(part 1 of 2)
# Autodesk Inventor assembly: 1103 Robot - Base2
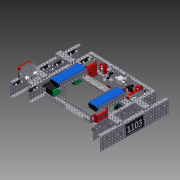
[picture p0: Inventor's stored thumbnail of the model, 180x180]
Saved by Autodesk Inventor 2012 (Build 160160000, 160)
## iProperties
Created: 2011-08-15
Part Number: 1103 Robot - Base2
Document SubType Name: Assembly
Designer: Dakota.Bayer
Author: Dakota.Bayer
## Documents named in this file (50)
- C:\Users\Wade\Documents\1103 Robot - CAD Assembly\1103 Chassis.iam
- C:\Users\Wade\Documents\1103 Robot - CAD Assembly\5 x 25.ipt
- C:\Users\Wade\Documents\1103 Robot - CAD Assembly\Flat Bearing Block.ipt
- C:\Users\Wade\Documents\1103 Robot - CAD Assembly\5 x 24.ipt
- C:\Users\Wade\Documents\1103 Robot - CAD Assembly\Bearing Block.iam
- C:\Users\Wade\Documents\1103 Robot - CAD Assembly\2 x 6.ipt
- C:\Users\Wade\Documents\1103 Robot - CAD Assembly\1103 Custom Chassis.ipt
- C:\Users\Wade\Documents\1103 Robot - CAD Assembly\2 x 25.ipt
- C:\Users\Wade\Documents\1103 Robot - CAD Assembly\4 Slotted Angle.ipt
- C:\Users\Wade\Documents\1103 Robot - CAD Assembly\4 x 6 cut.ipt
- C:\Users\Wade\Documents\1103 Robot - CAD Assembly\.5'' Screw & Nylock Nut.iam
- C:\Users\Wade\Documents\1103 Robot - CAD Assembly\2x .5'' Screw & Nylock Nut.iam
- C:\Users\Wade\Documents\24C VEX CAD Files\Screws & Nuts\Screw 8-32 x 0.500''-Silver.ipt
- C:\Users\Wade\Documents\24C VEX CAD Files\Screws & Nuts\Screw 6-32 x 0.500''-Silver.ipt
- C:\Users\Wade\Documents\24C VEX CAD Files\Screws & Nuts\Nut 8-32 Nylock.ipt
- C:\Users\Wade\Documents\24C VEX CAD Files\Washers & Spacers\Spacer (Nylon), 0.375''.ipt
- C:\Users\Wade\Documents\24C VEX CAD Files\Standoffs & Couplers\Standoff 0.50''.ipt
- C:\Users\Wade\Documents\24C VEX CAD Files\Screws & Nuts\Screw 8-32 x 0.250''-Silver.ipt
- C:\Users\Wade\Documents\24C VEX CAD Files\Screws & Nuts\Nut 8-32 Keps.ipt
- C:\Users\Wade\Documents\24C VEX CAD Files\Screws & Nuts\Screw 8-32 x 0.750''-Silver.ipt
- C:\Users\Wade\Documents\24C VEX CAD Files\Screws & Nuts\Screw 8-32 x 0.375''-Silver.ipt
- C:\Users\Wade\Documents\1103 Robot - CAD Assembly\.375'' Screw & Nylock Nut.iam
- C:\Users\Wade\Documents\24C VEX CAD Files\Motors & Sensors\2-Wire Motor 393-Without Wire.iam
- C:\Users\Wade\Documents\24C VEX CAD Files\Motors & Sensors\Ultrasonic Range Finder (Sensor).iam
- C:\Users\Wade\Documents\1103 Robot - CAD Assembly\VEX-HINGE-1 RevA_1.ipt
- C:\Users\Wade\Documents\1103 Robot - CAD Assembly\VEX-HINGE-PIN_1.ipt
- C:\Users\Wade\Documents\1103 Robot - CAD Assembly\VEX-HINGE-1 RevA 4x.ipt
- C:\Users\Wade\Documents\1103 Robot - CAD Assembly\VEX-HINGE-PIN 4x.ipt
- C:\Users\Wade\Documents\24C VEX CAD Files\Washers & Spacers\Spacer (Nylon), 0.125''.ipt
- C:\Users\Wade\Documents\1103 Robot - CAD Assembly\Drivetrain Encoder.iam
- C:\Users\Wade\Documents\24C VEX CAD Files\Motors & Sensors\Line Follower Sensor (Line Tracker)-Parts\Custom1x4 Mount.ipt
- C:\Users\Wade\Documents\24C VEX CAD Files\Other Parts\On-Off Switch.iam
- C:\Users\Wade\Documents\1103 Robot - CAD Assembly\5 x 25 Custom.ipt
- C:\Users\Wade\Documents\1103 Robot - CAD Assembly\Input Potentiometer.iam
- C:\Users\Wade\Documents\24C VEX CAD Files\Other Parts\Regulator Body.ipt
- C:\Users\Wade\Documents\24C VEX CAD Files\Other Parts\Regulator Nut.ipt
- C:\Users\Wade\Documents\24C VEX CAD Files\Other Parts\Tier Pump Fitting Nut.ipt
- C:\Users\Wade\Documents\24C VEX CAD Files\Other Parts\Tire Pump Fitting.ipt
- C:\Users\Wade\Documents\24C VEX CAD Files\Other Parts\Fitting for Cylinders.ipt
- C:\Users\Wade\Documents\24C VEX CAD Files\Metal Plates\Metal L (3x2) .ipt
- C:\Users\Wade\Documents\24C VEX CAD Files\Other Parts\Pneumatic Cylinder Mount.ipt
- C:\Users\Wade\Documents\1103 Robot - CAD Assembly\1103 ID Plate (with hardware).iam
- C:\Users\Wade\Documents\24C VEX CAD Files\Metal Plates\Plate 6x3.ipt
- C:\Users\Wade\Documents\24C VEX CAD Files\Metal C-Channels\Aluminum L-Channel 1x5x2.ipt
- C:\Users\Wade\Documents\24C VEX CAD Files\Metal Plates\Plate 4x3.ipt
- C:\Users\Wade\Documents\24C VEX CAD Files\Metal Angles\Angle 2x2x10.ipt
- C:\Users\Wade\Documents\24C VEX CAD Files\Other Parts\7.2V (Robot Battery) NiMH 3000mAh.ipt
- C:\Users\Wade\Documents\24C VEX CAD Files\Motors & Sensors\Line Follower Sensor (Line Tracker).iam
- C:\Users\Wade\Documents\24C VEX CAD Files\Washers & Spacers\Washer, Delrin.ipt
- C:\Users\Wade\Documents\24C VEX CAD Files\Screws & Nuts\Screw 8-32 x 0.875''-Silver.ipt
## Components (259 placed, 49 different names)
1. 5 x 25:2 — Mate:3, Mate:22, Mate:42, Mate:57, Mate:74, Flush:1, Flush:2, Flush:18, Flush:19, Mate:255, Flush:20, Flush:21, Flush:22, Flush:23, Flush:58, Flush:59, Mate:326, Mate:327, Mate:330, Mate:583, Mate:584, Angle:6, Mate:599, Mate:600, Mate:699
2. Flat Bearing Block:1 — Mate:3, Mate:324, Mate:325, Mate:698
3. .5'' Screw & Nylock Nut:3 [sub-assembly] — Mate:327, Mate:328
4. Flat Bearing Block:2 — Mate:22, Mate:328, Mate:329
5. Screw 8-32 x 0.500''-Silver:1 — Mate:366
6. Flat Bearing Block:3 — Mate:42, Mate:356, Mate:357
7. Screw 8-32 x 0.500''-Silver:2 — Mate:367
8. Screw 8-32 x 0.500''-Silver:3 — Mate:365
9. Flat Bearing Block:4 — Mate:57, Mate:358, Mate:359
10. Screw 8-32 x 0.500''-Silver:4 — Mate:364
11. Screw 8-32 x 0.500''-Silver:5 — Mate:363
12. Flat Bearing Block:5 — Mate:74, Mate:360, Mate:361
13. Screw 8-32 x 0.500''-Silver:6 — Mate:362
14. 5 x 24:1 — Flush:1, Flush:2, Mate:98, Mate:99, Mate:104, Mate:109, Mate:121, Flush:3, Flush:4, Mate:253, Mate:254, Mate:318, Flush:58, Flush:59, Mate:322, Tangent:152, Tangent:153, Tangent:154, Tangent:155, Tangent:156, Mate:422, Tangent:186, Mate:432, Tangent:190, Tangent:191, Mate:452, Flush:67, Mate:481, Mate:482, Flush:68, Mate:485, Tangent:220, Mate:598, Flush:555, Flush:556, Mate:695, Mate:696, Mate:697, Mate:701, Mate:703, Mate:704, Mate:705, Mate:706
15. Bearing Block:1 [sub-assembly] — Mate:98, Tangent:152, Tangent:153, Tangent:154
16. Flat Bearing Block:7 — Mate:99, Mate:319, Mate:320, Mate:323, Mate:695, Mate:696, Mate:698, Mate:700
17. Flat Bearing Block:8 — Mate:104, Mate:478, Mate:479, Mate:702
18. Screw 6-32 x 0.500''-Silver:2 — Mate:703, Mate:704, Mate:707
19. Screw 6-32 x 0.500''-Silver:3
20. Screw 6-32 x 0.500''-Silver:4
21. Flat Bearing Block:9 — Mate:109
22. 2-Wire Motor 393-Without Wire:1 [sub-assembly]
23. 2-Wire Motor 393-Without Wire:2 [sub-assembly] — Mate:478, Mate:480, Mate:702, Mate:707
24. 5 x 25 Custom:1 — Mate:121, Flush:3, Flush:4, Mate:122, Flush:5, Flush:6, Mate:430, Tangent:187, Mate:431, Tangent:188, Tangent:189, Mate:483, Mate:489, Mate:511, Mate:512, Mate:523, Angle:2, Mate:525, Mate:526, Mate:527, Mate:528, Mate:529, Mate:530, Mate:531, Mate:532, Mate:535, Mate:536, Angle:3, Mate:538, Mate:539, Mate:540, Mate:542, Angle:4, Flush:71, Mate:545, Flush:546, Mate:546, Flush:547, Flush:548, Mate:551, Mate:553, Mate:574, Mate:576, Mate:682, Angle:10, Mate:732
25. 5 x 24:2 — Mate:122, Flush:5, Flush:6, Mate:123, Mate:133, Mate:139, Flush:7, Flush:8, Mate:242, Mate:244, Mate:250, Flush:34, Flush:57, Tangent:157, Tangent:158, Tangent:159, Tangent:160, Tangent:161, Tangent:162, Mate:333, Mate:433, Tangent:192, Tangent:193, Mate:486, Tangent:221, Tangent:222, Tangent:223, Mate:488, Mate:514, Mate:515, Mate:516, Mate:518, Flush:553, Mate:596, Flush:554, Angle:7, Mate:708, Mate:709, Mate:710, Mate:711
26. .5'' Screw & Nylock Nut:5 [sub-assembly] — Mate:332, Mate:333
27. Screw 8-32 x 0.500''-Silver:8 — Mate:335
28. Flat Bearing Block:10 — Mate:123, Mate:332, Mate:334, Mate:700
29. Flat Bearing Block:11 — Mate:250
30. Screw 6-32 x 0.500''-Silver:5
31. Screw 6-32 x 0.500''-Silver:6
32. Bearing Block:2 [sub-assembly] — Mate:133, Tangent:157, Tangent:158, Tangent:159
33. Flat Bearing Block:12 — Mate:244, Mate:712
34. Screw 6-32 x 0.500''-Silver:7 — Mate:708, Mate:709
35. Bearing Block:3 [sub-assembly] — Mate:139, Tangent:160, Tangent:161, Tangent:162
36. 2-Wire Motor 393-Without Wire:3 [sub-assembly] — Mate:249, Mate:712
37. 2-Wire Motor 393-Without Wire:4 [sub-assembly]
38. 5 x 25:4 — Flush:7, Flush:8, Mate:207, Mate:213, Mate:219, Mate:224, Mate:229, Mate:241, Rotation:2, Flush:56, Mate:581, Mate:582, Angle:5, Mate:585
39. Screw 8-32 x 0.500''-Silver:9 — Mate:354
40. Screw 8-32 x 0.500''-Silver:10 — Mate:355
41. Flat Bearing Block:13 — Mate:207, Mate:352, Mate:353
42. Screw 8-32 x 0.500''-Silver:11 — Mate:346
43. Screw 8-32 x 0.500''-Silver:12 — Mate:347
44. Flat Bearing Block:14 — Mate:213, Mate:344, Mate:345
45. Screw 8-32 x 0.500''-Silver:13 — Mate:350
46. Screw 8-32 x 0.500''-Silver:14 — Mate:351
47. Flat Bearing Block:15 — Mate:219, Rotation:2, Mate:348, Mate:349
48. Screw 8-32 x 0.500''-Silver:15 — Mate:342
49. Screw 8-32 x 0.500''-Silver:16 — Mate:343
50. Flat Bearing Block:16 — Mate:224, Mate:340, Mate:341
51. Screw 8-32 x 0.500''-Silver:17 — Mate:336
52. Screw 8-32 x 0.500''-Silver:18 — Mate:337
53. Flat Bearing Block:17 — Mate:229, Mate:338, Mate:339
54. Standoff 0.50'':1 — Mate:381
55. Standoff 0.50'':2 — Mate:383
56. Standoff 0.50'':3 — Mate:380
57. Standoff 0.50'':4 — Mate:382
58. Standoff 0.50'':5 — Mate:372
59. Standoff 0.50'':6 — Mate:374
60. Standoff 0.50'':7 — Mate:375
61. Standoff 0.50'':8 — Mate:373
62. 2 x 6:1 — Mate:255, Flush:20, Flush:21, Mate:368, Mate:369
63. 2 x 6:2 — Mate:254, Flush:18, Flush:19, Mate:370, Mate:371
64. 2 x 6:3 — Mate:241, Flush:57, Mate:378, Mate:379
65. 2 x 6:4 — Mate:242, Mate:376, Mate:377
66. Screw 6-32 x 0.500''-Silver:8 — Mate:249, Mate:710, Mate:711
67. 1103 Custom Chassis:1 — Mate:253, Flush:22, Flush:23, Flush:56, Tangent:171, Tangent:172, Mate:423, Tangent:173, Tangent:174, Mate:424, Mate:425, Tangent:175, Tangent:176, Tangent:177, Mate:426, Mate:427, Tangent:178, Tangent:179, Tangent:180, Tangent:181, Mate:428, Mate:429, Tangent:182, Tangent:183, Tangent:184, Tangent:185, Tangent:207, Mate:611, Flush:557, Flush:558, Mate:612, Flush:559, Flush:560, Mate:613, Mate:614, Mate:615, Mate:616, Mate:617, Mate:618, Mate:619, Mate:621, Mate:622, Mate:623, Mate:624
68. 2 x 25:1 — Flush:34, Mate:434, Mate:435, Flush:62, Flush:63, Flush:64, Flush:65, Mate:448, Mate:449, Tangent:199, Tangent:200, Tangent:201, Tangent:202, Mate:450, Mate:451, Tangent:203, Tangent:204, Tangent:205, Tangent:206, Mate:452, Flush:67, Mate:453, Mate:456, Mate:457, Mate:458, Mate:459, Mate:468, Mate:469, Mate:470, Mate:471, Mate:472
69. Standoff 0.50'':9 — Mate:386
70. Standoff 0.50'':10 — Mate:387
71. 4 Slotted Angle:1 — Mate:384, Mate:385, Mate:418, Mate:419
72. Spacer (Nylon), 0.375'':1 — Mate:416
73. Spacer (Nylon), 0.375'':2 — Mate:417
74. 4 x 6 cut:1 — Mate:414, Mate:415
75. Ultrasonic Range Finder (Sensor):1 [sub-assembly]
76. Standoff 0.50'':11 — Mate:390
77. Standoff 0.50'':12 — Mate:391
78. 4 Slotted Angle:2 — Mate:388, Mate:389, Mate:410, Mate:411
79. Spacer (Nylon), 0.375'':3 — Mate:408
80. Spacer (Nylon), 0.375'':4 — Mate:409
81. 4 x 6 cut:2 — Mate:406, Mate:407
82. Ultrasonic Range Finder (Sensor):2 [sub-assembly]
83. Bearing Block:4 [sub-assembly] — Mate:318, Tangent:155, Tangent:156, Mate:701
84. .5'' Screw & Nylock Nut:1 [sub-assembly] — Mate:319, Mate:320
85. .5'' Screw & Nylock Nut:2 [sub-assembly] — Mate:322, Mate:323, Mate:697
86. 2x .5'' Screw & Nylock Nut:1 [sub-assembly] — Mate:324, Mate:325, Mate:326, Mate:699
87. .5'' Screw & Nylock Nut:4 [sub-assembly] — Mate:329, Mate:330
88. Nut 8-32 Nylock:1 — Mate:334, Mate:335
89. Nut 8-32 Nylock:2 — Mate:336, Mate:338
90. Nut 8-32 Nylock:3 — Mate:337, Mate:339
91. Nut 8-32 Nylock:4 — Mate:340, Mate:342
92. Nut 8-32 Nylock:5 — Mate:341, Mate:343
93. Nut 8-32 Nylock:6 — Mate:345, Mate:347
94. Nut 8-32 Nylock:7 — Mate:344, Mate:346
95. Nut 8-32 Nylock:8 — Mate:348, Mate:351
96. Nut 8-32 Nylock:9 — Mate:349, Mate:350
97. Nut 8-32 Nylock:10 — Mate:352, Mate:355
98. Nut 8-32 Nylock:11 — Mate:353, Mate:354
99. Nut 8-32 Nylock:12 — Mate:356, Mate:366
100. Nut 8-32 Nylock:13 — Mate:357, Mate:367
101. Nut 8-32 Nylock:14 — Mate:358, Mate:364
102. Nut 8-32 Nylock:15 — Mate:359, Mate:365
103. Nut 8-32 Nylock:16 — Mate:361, Mate:363
104. Nut 8-32 Nylock:17 — Mate:360, Mate:362
105. Screw 8-32 x 0.250''-Silver:1 — Mate:368, Mate:372
106. Screw 8-32 x 0.250''-Silver:2 — Mate:369, Mate:373
107. Screw 8-32 x 0.250''-Silver:3 — Mate:371, Mate:375
108. Screw 8-32 x 0.250''-Silver:4 — Mate:370, Mate:374
109. Screw 8-32 x 0.250''-Silver:5 — Mate:379, Mate:381
110. Screw 8-32 x 0.250''-Silver:6 — Mate:378, Mate:380
111. Screw 8-32 x 0.250''-Silver:7 — Mate:377, Mate:382
112. Screw 8-32 x 0.250''-Silver:8 — Mate:376, Mate:383
113. Screw 8-32 x 0.250''-Silver:9 — Mate:384, Mate:386
114. Screw 8-32 x 0.250''-Silver:10 — Mate:385, Mate:387
115. Screw 8-32 x 0.250''-Silver:11 — Mate:388, Mate:391
116. Screw 8-32 x 0.250''-Silver:12 — Mate:389, Mate:390
117. Screw 8-32 x 0.375''-Silver:2
118. Screw 8-32 x 0.375''-Silver:1
119. Nut 8-32 Keps:1
120. Nut 8-32 Keps:2
121. Nut 8-32 Keps:3
122. Screw 8-32 x 0.375''-Silver:4
123. Nut 8-32 Keps:4
124. Screw 8-32 x 0.375''-Silver:3
125. Screw 8-32 x 0.750''-Silver:1 — Mate:406, Mate:408, Mate:413
126. Screw 8-32 x 0.750''-Silver:2 — Mate:407, Mate:409, Mate:412
127. Nut 8-32 Nylock:18 — Mate:410, Mate:413
128. Nut 8-32 Nylock:19 — Mate:411, Mate:412
129. Screw 8-32 x 0.750''-Silver:3 — Mate:414, Mate:416, Mate:421
130. Screw 8-32 x 0.750''-Silver:4 — Mate:415, Mate:417, Mate:420
131. Nut 8-32 Nylock:20 — Mate:418, Mate:421
132. Nut 8-32 Nylock:21 — Mate:419, Mate:420
133. .375'' Screw & Nylock Nut:1 [sub-assembly] — Tangent:171, Tangent:172, Mate:422
134. .375'' Screw & Nylock Nut:2 [sub-assembly] — Mate:425, Tangent:175, Tangent:176
135. .375'' Screw & Nylock Nut:3 [sub-assembly] — Mate:423, Tangent:173, Tangent:174
136. .375'' Screw & Nylock Nut:4 [sub-assembly] — Mate:424, Tangent:177, Tangent:207
137. .375'' Screw & Nylock Nut:5 [sub-assembly] — Mate:426, Tangent:178, Tangent:179
138. .375'' Screw & Nylock Nut:6 [sub-assembly] — Mate:427, Tangent:180, Tangent:181
139. .375'' Screw & Nylock Nut:7 [sub-assembly] — Mate:428, Tangent:184, Tangent:185
140. .375'' Screw & Nylock Nut:8 [sub-assembly] — Mate:429, Tangent:182, Tangent:183
141. .375'' Screw & Nylock Nut:9 [sub-assembly] — Mate:430, Tangent:186, Tangent:187
142. .375'' Screw & Nylock Nut:10 [sub-assembly] — Mate:431, Tangent:188, Tangent:189
143. .375'' Screw & Nylock Nut:11 [sub-assembly] — Mate:432, Tangent:190, Tangent:191
144. .375'' Screw & Nylock Nut:12 [sub-assembly] — Mate:433, Tangent:192, Tangent:193
145. VEX-HINGE-1 RevA_1:1 — Mate:434, Mate:437, Flush:60, Flush:62, Flush:63, Flush:66, Tangent:210, Tangent:211, Tangent:212, Tangent:213, Tangent:214, Tangent:215, Mate:464, Mate:465, Mate:466
146. VEX-HINGE-PIN_1:1 — Mate:437, Flush:60
147. VEX-HINGE-1 RevA 4x:1 — Mate:435, Mate:436, Flush:61, Flush:64, Flush:65, Tangent:208, Tangent:209, Mate:455, Tangent:216, Tangent:217, Mate:467
148. VEX-HINGE-PIN 4x:1 — Mate:436, Flush:61
149. Screw 8-32 x 0.500''-Silver:23 — Mate:463, Mate:464, Mate:473
150. Screw 8-32 x 0.500''-Silver:21 — Mate:461, Mate:466, Mate:475
151. Screw 8-32 x 0.500''-Silver:20 — Mate:460, Mate:467, Mate:476
152. Screw 8-32 x 0.500''-Silver:22 — Mate:462, Mate:465, Mate:474
153. Screw 8-32 x 0.500''-Silver:19 — Mate:454, Mate:455, Mate:477
154. .375'' Screw & Nylock Nut:18 [sub-assembly] — Mate:448, Tangent:199, Tangent:200
155. .375'' Screw & Nylock Nut:19 [sub-assembly] — Mate:449, Tangent:201, Tangent:202
156. .375'' Screw & Nylock Nut:20 [sub-assembly] — Mate:450, Tangent:203, Tangent:204
157. .375'' Screw & Nylock Nut:21 [sub-assembly] — Mate:451, Tangent:205, Tangent:206
158. Spacer (Nylon), 0.125'':1 — Mate:453, Tangent:208, Tangent:209, Mate:454
159. Spacer (Nylon), 0.125'':2 — Mate:456, Tangent:216, Tangent:217, Mate:460
160. Spacer (Nylon), 0.125'':3 — Mate:457, Tangent:214, Tangent:215, Mate:461
161. Spacer (Nylon), 0.125'':4 — Mate:458, Tangent:212, Tangent:213, Mate:462
162. Spacer (Nylon), 0.125'':5 — Mate:459, Tangent:210, Tangent:211, Mate:463
163. Nut 8-32 Nylock:22 — Mate:468, Mate:473
164. Nut 8-32 Nylock:23 — Mate:469, Mate:474
165. Nut 8-32 Nylock:24 — Mate:470, Mate:475
166. Nut 8-32 Nylock:25 — Mate:471, Mate:476
167. Nut 8-32 Nylock:26 — Mate:472, Mate:477
168. Screw 6-32 x 0.500''-Silver:9 — Mate:479, Mate:480, Mate:481, Mate:705, Mate:706
169. Drivetrain Encoder:1 [sub-assembly] — Mate:482, Flush:68, Mate:483, Mate:484
170. Drivetrain Encoder:2 [sub-assembly] — Mate:487, Mate:488, Mate:489
171. Bearing Block:5 [sub-assembly] — Mate:484, Mate:485, Tangent:220
172. Bearing Block:6 [sub-assembly] — Mate:486, Tangent:221, Tangent:222, Tangent:223, Mate:487
173. Screw 8-32 x 0.250''-Silver:13 — Mate:509, Mate:510, Mate:682
174. Screw 8-32 x 0.375''-Silver:5 — Mate:507, Mate:681, Mate:687, Mate:731
175. Screw 8-32 x 0.375''-Silver:6 — Mate:504, Mate:683, Mate:684, Mate:686, Mate:729
176. Screw 8-32 x 0.375''-Silver:7 — Mate:503, Mate:688, Mate:690, Mate:730
177. Nut 8-32 Nylock:27 — Mate:504, Mate:505, Mate:683, Mate:685
178. Nut 8-32 Nylock:28 — Mate:503, Mate:506, Mate:691
179. Custom1x4 Mount:1 — Mate:505, Mate:506, Mate:508, Mate:512, Mate:681, Mate:684, Mate:685, Mate:689, Mate:690, Mate:691, Mate:692, Mate:693
180. Line Follower Sensor (Line Tracker):1 [sub-assembly] — Mate:686, Mate:693, Angle:8, Mate:729
181. Line Follower Sensor (Line Tracker):2 [sub-assembly] — Mate:688, Mate:689, Angle:9, Mate:730, Mate:731
182. Line Follower Sensor (Line Tracker):3 [sub-assembly] — Mate:687, Mate:692, Angle:8, Angle:9, Angle:10
183. Standoff 0.50'':13 — Mate:507, Mate:508, Mate:509, Mate:510, Mate:511
184. Line Follower Sensor (Line Tracker):4 [sub-assembly] — Mate:679, Mate:680, Angle:7
185. Screw 8-32 x 0.250''-Silver:14 — Mate:514, Mate:515, Mate:516, Mate:517
186. Standoff 0.50'':14 — Mate:517, Mate:518, Mate:521, Mate:680
187. Screw 8-32 x 0.375''-Silver:8 — Mate:521, Mate:679
188. On-Off Switch:1 [sub-assembly] — Mate:523, Angle:2, Mate:732
189. Input Potentiometer:1 [sub-assembly] — Mate:525, Mate:527, Mate:528, Mate:529
190. Input Potentiometer:2 [sub-assembly] — Mate:526, Mate:530, Mate:531, Mate:532
191. Regulator Body:1 — Mate:535, Mate:537, Angle:3, Mate:538, Mate:544, Mate:694
192. Regulator Nut:1 — Mate:536, Mate:537
193. Tier Pump Fitting Nut:1 — Mate:541, Mate:542
194. Tire Pump Fitting:1 — Mate:539, Mate:540, Mate:541, Angle:4
195. Fitting for Cylinders:1 — Mate:544, Mate:694
196. Metal L (3x2) :1 — Flush:71, Mate:545, Flush:546, Mate:554, Mate:555, Mate:560, Flush:551, Flush:552, Mate:573
197. Metal L (3x2) :2 — Mate:546, Flush:547, Flush:548, Mate:550, Mate:552, Mate:559, Flush:549, Flush:550, Mate:575
198. .375'' Screw & Nylock Nut:22 [sub-assembly] — Mate:553, Mate:554, Mate:555
199. .375'' Screw & Nylock Nut:24 [sub-assembly] — Mate:550, Mate:551, Mate:552
200. Pneumatic Cylinder Mount:1 — Mate:559, Flush:549, Flush:550, Mate:567, Mate:568, Mate:569, Mate:570, Mate:571, Mate:572, Mate:717, Mate:718, Mate:719, Mate:721, Mate:722, Mate:724
201. Pneumatic Cylinder Mount:2 — Mate:560, Flush:551, Flush:552, Mate:561, Mate:562, Mate:566, Mate:713, Mate:714, Mate:715, Mate:725, Mate:727, Mate:728
202. Screw 8-32 x 0.500''-Silver:25 — Mate:567, Mate:568, Mate:571, Mate:578
203. Screw 8-32 x 0.375''-Silver:9 — Mate:579
204. Screw 8-32 x 0.500''-Silver:27 — Mate:561, Mate:562, Mate:566, Mate:580
205. Screw 8-32 x 0.375''-Silver:10 — Mate:569, Mate:570, Mate:572, Mate:577
206. Nut 8-32 Nylock:29 — Mate:573, Mate:579
207. Nut 8-32 Nylock:30 — Mate:574, Mate:580
208. Nut 8-32 Nylock:31 — Mate:575, Mate:577
209. Nut 8-32 Nylock:32 — Mate:576, Mate:578
210. 1103 ID Plate (with hardware):1 [sub-assembly] — Mate:581, Mate:582, Angle:5
211. 1103 ID Plate (with hardware):2 [sub-assembly] — Mate:583, Mate:584, Angle:6
212. Plate 6x3:1 — Mate:585, Flush:553, Flush:554, Mate:586, Mate:587, Mate:588, Mate:589, Mate:590, Mate:591, Mate:592, Mate:594, Mate:595, Mate:597, Mate:593
213. .375'' Screw & Nylock Nut:25 [sub-assembly] — Mate:586, Mate:587, Mate:588
214. .375'' Screw & Nylock Nut:26 [sub-assembly] — Mate:589, Mate:590, Mate:591
215. .375'' Screw & Nylock Nut:27 [sub-assembly] — Mate:595, Mate:596, Mate:597
216. .375'' Screw & Nylock Nut:28 [sub-assembly] — Mate:592, Mate:593, Mate:594
217. Plate 6x3:2 — Mate:598, Flush:555, Flush:556, Mate:601, Mate:602, Mate:603, Mate:604, Mate:605, Mate:606, Mate:607, Mate:608, Mate:609, Mate:610
218. .375'' Screw & Nylock Nut:29 [sub-assembly] — Mate:599, Mate:600, Mate:601
219. .375'' Screw & Nylock Nut:30 [sub-assembly] — Mate:602, Mate:603, Mate:604
220. .375'' Screw & Nylock Nut:31 [sub-assembly] — Mate:608, Mate:609, Mate:610
221. .375'' Screw & Nylock Nut:32 [sub-assembly] — Mate:605, Mate:606, Mate:607
222. Aluminum L-Channel 1x5x2:1 — Mate:611, Flush:557, Flush:558, Flush:561, Mate:625, Flush:562, Mate:667, Mate:668
223. Aluminum L-Channel 1x5x2:2 — Mate:612, Flush:559, Flush:560, Mate:620, Mate:626, Flush:627, Flush:628, Mate:669, Mate:670, Mate:677, Mate:678
224. .375'' Screw & Nylock Nut:33 [sub-assembly] — Mate:613, Mate:614, Mate:615
225. .375'' Screw & Nylock Nut:34 [sub-assembly] — Mate:616, Mate:617, Mate:618
226. .375'' Screw & Nylock Nut:35 [sub-assembly] — Mate:619, Mate:620, Mate:621
227. .375'' Screw & Nylock Nut:36 [sub-assembly] — Mate:622, Mate:623, Mate:624
228. Plate 4x3:1 — Flush:561, Mate:625, Flush:562, Mate:627, Flush:629, Flush:630, Mate:628, Flush:631, Flush:632, Mate:663
229. Plate 4x3:2 — Mate:626, Flush:627, Flush:628, Mate:629, Flush:633, Flush:634, Mate:630, Flush:635, Flush:636, Mate:641
230. Angle 2x2x10:1 — Mate:627, Flush:629, Flush:630, Mate:631, Mate:632, Mate:633, Mate:646, Mate:647, Mate:648, Mate:656, Flush:637, Mate:659, Mate:660, Mate:661, Mate:662, Mate:664
231. Angle 2x2x10:2 — Mate:628, Flush:631, Flush:632, Mate:634, Mate:635, Mate:636, Mate:643, Mate:644, Mate:645, Mate:655
232. Angle 2x2x10:3 — Mate:629, Flush:633, Flush:634, Mate:637, Mate:638, Mate:639, Mate:649, Mate:650, Mate:651
233. Angle 2x2x10:4 — Mate:630, Flush:635, Flush:636, Mate:640, Mate:642, Mate:652, Mate:653, Mate:654, Mate:657, Mate:658, Flush:638, Mate:671, Mate:672, Mate:673, Mate:674
234. .375'' Screw & Nylock Nut:37 [sub-assembly] — Mate:631, Mate:632, Mate:633
235. .375'' Screw & Nylock Nut:38 [sub-assembly] — Mate:634, Mate:635, Mate:636
236. .375'' Screw & Nylock Nut:39 [sub-assembly] — Mate:637, Mate:638, Mate:639
237. .375'' Screw & Nylock Nut:40 [sub-assembly] — Mate:640, Mate:641, Mate:642
238. .375'' Screw & Nylock Nut:41 [sub-assembly] — Mate:646, Mate:647, Mate:648
239. .375'' Screw & Nylock Nut:42 [sub-assembly] — Mate:643, Mate:644, Mate:645
240. .375'' Screw & Nylock Nut:43 [sub-assembly] — Mate:652, Mate:653, Mate:654
241. .375'' Screw & Nylock Nut:44 [sub-assembly] — Mate:649, Mate:650, Mate:651
242. 7.2V (Robot Battery) NiMH 3000mAh:1 — Mate:655, Mate:656, Flush:637
243. 7.2V (Robot Battery) NiMH 3000mAh:2 — Mate:657, Mate:658, Flush:638
244. Screw 8-32 x 0.375''-Silver:11 — Mate:659, Mate:660, Mate:661, Mate:666
245. Screw 8-32 x 0.375''-Silver:12 — Mate:662, Mate:663, Mate:664, Mate:665
246. Nut 8-32 Nylock:33 — Mate:666, Mate:667
247. Nut 8-32 Nylock:34 — Mate:665, Mate:668
248. Screw 8-32 x 0.375''-Silver:13 — Mate:672, Mate:673, Mate:674, Mate:676
249. Nut 8-32 Nylock:35 — Mate:675, Mate:677
250. Screw 8-32 x 0.375''-Silver:14 — Mate:669, Mate:670, Mate:671, Mate:675
251. Nut 8-32 Nylock:36 — Mate:676, Mate:678
252. Washer, Delrin:1 — Mate:713, Mate:715, Mate:716
253. Washer, Delrin:2 — Mate:714, Mate:716
254. Washer, Delrin:3 — Mate:718, Mate:719, Mate:720
255. Washer, Delrin:4 — Mate:717, Mate:720
256. Nut 8-32 Nylock:37 — Mate:723, Mate:724
257. Screw 8-32 x 0.875''-Silver:1 — Mate:721, Mate:722, Mate:723
258. Nut 8-32 Nylock:38 — Mate:726, Mate:727
259. Screw 8-32 x 0.875''-Silver:2 — Mate:725, Mate:726, Mate:728
## Relationships (704: Mate 477, Tangent 157, Flush 60, Angle 9, RelateRotation 1)
- Mate:3: 5 x 25:2 ↔ Flat Bearing Block:1
- Mate:22: 5 x 25:2 ↔ Flat Bearing Block:2
- [Mate]: 5 x 25:2 ↔ Screw 8-32 x 0.500''-Silver:2
- [Tangent] (0.2286 mm): 5 x 25:2 ↔ Screw 8-32 x 0.500''-Silver:2
- [Tangent] (0.2286 mm): 5 x 25:2 ↔ Screw 8-32 x 0.500''-Silver:2
- [Mate]: 5 x 25:2 ↔ Screw 8-32 x 0.500''-Silver:1
- [Tangent] (0.2286 mm): 5 x 25:2 ↔ Screw 8-32 x 0.500''-Silver:1
- [Tangent] (0.2286 mm): 5 x 25:2 ↔ Screw 8-32 x 0.500''-Silver:1
- Mate:42: 5 x 25:2 ↔ Flat Bearing Block:3
- [Mate]: Screw 8-32 x 0.500''-Silver:1 ↔ Flat Bearing Block:3
- [Mate]: Flat Bearing Block:3 ↔ Screw 8-32 x 0.500''-Silver:2
- Mate:57: 5 x 25:2 ↔ Flat Bearing Block:4
- [Mate]: 5 x 25:2 ↔ Screw 8-32 x 0.500''-Silver:4
- [Tangent] (0.2286 mm): 5 x 25:2 ↔ Screw 8-32 x 0.500''-Silver:4
- [Tangent] (0.2286 mm): 5 x 25:2 ↔ Screw 8-32 x 0.500''-Silver:4
- [Mate]: 5 x 25:2 ↔ Screw 8-32 x 0.500''-Silver:3
- [Tangent] (0.2286 mm): 5 x 25:2 ↔ Screw 8-32 x 0.500''-Silver:3
- [Tangent] (0.2286 mm): 5 x 25:2 ↔ Screw 8-32 x 0.500''-Silver:3
- [Mate]: Flat Bearing Block:4 ↔ Screw 8-32 x 0.500''-Silver:4
- [Mate]: Screw 8-32 x 0.500''-Silver:3 ↔ Flat Bearing Block:4
- Mate:74: 5 x 25:2 ↔ Flat Bearing Block:5
- [Mate] (-1.524 mm): 5 x 25:2 ↔ Screw 8-32 x 0.500''-Silver:5
- [Tangent] (0.2286 mm): 5 x 25:2 ↔ Screw 8-32 x 0.500''-Silver:5
- [Tangent] (0.2286 mm): 5 x 25:2 ↔ Screw 8-32 x 0.500''-Silver:5
- [Mate] (-1.524 mm): 5 x 25:2 ↔ Screw 8-32 x 0.500''-Silver:6
- [Tangent] (0.2286 mm): 5 x 25:2 ↔ Screw 8-32 x 0.500''-Silver:6
- [Tangent] (0.2286 mm): 5 x 25:2 ↔ Screw 8-32 x 0.500''-Silver:6
- [Mate]: Screw 8-32 x 0.500''-Silver:5 ↔ Flat Bearing Block:5
- [Mate]: Flat Bearing Block:5 ↔ Screw 8-32 x 0.500''-Silver:6
- Flush:1: 5 x 25:2 ↔ 5 x 24:1
- Flush:2: 5 x 25:2 ↔ 5 x 24:1
- Mate:98: 5 x 24:1 ↔ Bearing Block:1
- Mate:99: 5 x 24:1 ↔ Flat Bearing Block:7
- Mate:104: 5 x 24:1 ↔ Flat Bearing Block:8
- [Mate]: 5 x 24:1 ↔ Screw 6-32 x 0.500''-Silver:2
- Mate:109: 5 x 24:1 ↔ Flat Bearing Block:9
- [Mate]: 5 x 24:1 ↔ Screw 6-32 x 0.500''-Silver:3
- [Mate]: 5 x 24:1 ↔ Screw 6-32 x 0.500''-Silver:4
- [Mate]: Screw 6-32 x 0.500''-Silver:3 ↔ Flat Bearing Block:9
- [Mate]: Screw 6-32 x 0.500''-Silver:4 ↔ Flat Bearing Block:9
- [Mate]: Flat Bearing Block:9 ↔ 2-Wire Motor 393-Without Wire:1
- [Mate]: Screw 6-32 x 0.500''-Silver:3 ↔ 2-Wire Motor 393-Without Wire:1
- [Mate]: Screw 6-32 x 0.500''-Silver:4 ↔ 2-Wire Motor 393-Without Wire:1
- [Mate]: Flat Bearing Block:8 ↔ 2-Wire Motor 393-Without Wire:2
- Mate:121: 5 x 24:1 ↔ 5 x 25 Custom:1
- Flush:3: 5 x 24:1 ↔ 5 x 25 Custom:1
- Flush:4: 5 x 24:1 ↔ 5 x 25 Custom:1
- Mate:122: 5 x 25 Custom:1 ↔ 5 x 24:2
- Flush:5: 5 x 25 Custom:1 ↔ 5 x 24:2
- Flush:6: 5 x 25 Custom:1 ↔ 5 x 24:2
- Mate:123: 5 x 24:2 ↔ Flat Bearing Block:10
- [Tangent] (0.2286 mm): 5 x 24:2 ↔ Screw 8-32 x 0.500''-Silver:8
- [Tangent] (0.2286 mm): 5 x 24:2 ↔ Screw 8-32 x 0.500''-Silver:8
- [Mate]: Screw 8-32 x 0.500''-Silver:8 ↔ Flat Bearing Block:10
- [Mate]: 5 x 24:2 ↔ Screw 6-32 x 0.500''-Silver:6
- [Mate]: 5 x 24:2 ↔ Screw 6-32 x 0.500''-Silver:5
- [Mate]: Flat Bearing Block:11 ↔ Screw 6-32 x 0.500''-Silver:5
- [Mate]: Flat Bearing Block:11 ↔ Screw 6-32 x 0.500''-Silver:6
- Mate:133: 5 x 24:2 ↔ Bearing Block:2
- [Mate]: 5 x 24:2 ↔ Screw 6-32 x 0.500''-Silver:7
- Mate:139: 5 x 24:2 ↔ Bearing Block:3
- [Mate]: Flat Bearing Block:12 ↔ 2-Wire Motor 393-Without Wire:3
- [Mate]: Flat Bearing Block:11 ↔ 2-Wire Motor 393-Without Wire:4
- Flush:7: 5 x 24:2 ↔ 5 x 25:4
- Flush:8: 5 x 24:2 ↔ 5 x 25:4
- Mate:207: 5 x 25:4 ↔ Flat Bearing Block:13
- [Mate]: 5 x 25:4 ↔ Screw 8-32 x 0.500''-Silver:9
- [Tangent] (0.2286 mm): 5 x 25:4 ↔ Screw 8-32 x 0.500''-Silver:9
- [Tangent] (0.2286 mm): 5 x 25:4 ↔ Screw 8-32 x 0.500''-Silver:9
- [Mate]: 5 x 25:4 ↔ Screw 8-32 x 0.500''-Silver:10
- [Tangent] (0.2286 mm): 5 x 25:4 ↔ Screw 8-32 x 0.500''-Silver:10
- [Tangent] (0.2286 mm): 5 x 25:4 ↔ Screw 8-32 x 0.500''-Silver:10
- [Mate]: Screw 8-32 x 0.500''-Silver:9 ↔ Flat Bearing Block:13
- [Mate]: Screw 8-32 x 0.500''-Silver:10 ↔ Flat Bearing Block:13
- [Mate]: 5 x 25:4 ↔ Screw 8-32 x 0.500''-Silver:11
- Mate:213: 5 x 25:4 ↔ Flat Bearing Block:14
- [Mate]: 5 x 25:4 ↔ Screw 8-32 x 0.500''-Silver:12
- [Tangent] (0.2286 mm): 5 x 25:4 ↔ Screw 8-32 x 0.500''-Silver:11
- [Tangent] (0.2286 mm): 5 x 25:4 ↔ Screw 8-32 x 0.500''-Silver:11
- [Tangent] (0.2286 mm): 5 x 25:4 ↔ Screw 8-32 x 0.500''-Silver:12
- [Tangent] (0.2286 mm): 5 x 25:4 ↔ Screw 8-32 x 0.500''-Silver:12
- [Mate]: Screw 8-32 x 0.500''-Silver:11 ↔ Flat Bearing Block:14
- [Mate]: Screw 8-32 x 0.500''-Silver:12 ↔ Flat Bearing Block:14
- [Mate] (-1.524 mm): 5 x 25:4 ↔ Screw 8-32 x 0.500''-Silver:13
- [Mate] (-1.524 mm): 5 x 25:4 ↔ Screw 8-32 x 0.500''-Silver:14
- Mate:219: 5 x 25:4 ↔ Flat Bearing Block:15
- [Tangent] (0.2286 mm): 5 x 25:4 ↔ Screw 8-32 x 0.500''-Silver:13
- [Tangent] (0.2286 mm): 5 x 25:4 ↔ Screw 8-32 x 0.500''-Silver:13
- [Tangent] (0.2286 mm): 5 x 25:4 ↔ Screw 8-32 x 0.500''-Silver:14
- [Tangent] (0.2286 mm): 5 x 25:4 ↔ Screw 8-32 x 0.500''-Silver:14
- [Mate]: Screw 8-32 x 0.500''-Silver:13 ↔ Flat Bearing Block:15
- [Mate]: Screw 8-32 x 0.500''-Silver:14 ↔ Flat Bearing Block:15
- [Mate]: 5 x 25:4 ↔ Screw 8-32 x 0.500''-Silver:15
- [Mate]: 5 x 25:4 ↔ Screw 8-32 x 0.500''-Silver:16
- Mate:224: 5 x 25:4 ↔ Flat Bearing Block:16
- [Tangent] (0.2286 mm): 5 x 25:4 ↔ Screw 8-32 x 0.500''-Silver:15
- [Tangent] (0.2286 mm): 5 x 25:4 ↔ Screw 8-32 x 0.500''-Silver:15
- [Tangent] (0.2286 mm): 5 x 25:4 ↔ Screw 8-32 x 0.500''-Silver:16
- [Tangent] (0.2286 mm): 5 x 25:4 ↔ Screw 8-32 x 0.500''-Silver:16
- [Mate]: Screw 8-32 x 0.500''-Silver:15 ↔ Flat Bearing Block:16
- [Mate]: Screw 8-32 x 0.500''-Silver:16 ↔ Flat Bearing Block:16
- [Mate]: 5 x 25:4 ↔ Screw 8-32 x 0.500''-Silver:18
- [Mate]: 5 x 25:4 ↔ Screw 8-32 x 0.500''-Silver:17
- Mate:229: 5 x 25:4 ↔ Flat Bearing Block:17
- [Tangent] (0.2286 mm): 5 x 25:4 ↔ Screw 8-32 x 0.500''-Silver:17
- [Tangent] (0.2286 mm): 5 x 25:4 ↔ Screw 8-32 x 0.500''-Silver:17
- [Tangent] (0.2286 mm): 5 x 25:4 ↔ Screw 8-32 x 0.500''-Silver:18
- [Tangent] (0.2286 mm): 5 x 25:4 ↔ Screw 8-32 x 0.500''-Silver:18
- [Mate]: Screw 8-32 x 0.500''-Silver:17 ↔ Flat Bearing Block:17
- [Mate]: Screw 8-32 x 0.500''-Silver:18 ↔ Flat Bearing Block:17
- [Mate]: 5 x 25:4 ↔ Standoff 0.50'':1
- [Mate]: 5 x 25:4 ↔ Standoff 0.50'':3
- [Mate]: 5 x 25:2 ↔ Standoff 0.50'':6
- [Mate]: 5 x 24:1 ↔ Standoff 0.50'':7
- [Mate]: 5 x 24:1 ↔ Standoff 0.50'':5
- [Mate]: 5 x 25:2 ↔ Standoff 0.50'':8
- Mate:241: 5 x 25:4 ↔ 2 x 6:3
- Mate:242: 5 x 24:2 ↔ 2 x 6:4
- Mate:244: 5 x 24:2 ↔ Flat Bearing Block:12
- [Mate]: Flat Bearing Block:12 ↔ 2-Wire Motor 393-Without Wire:3
- [Mate]: Flat Bearing Block:12 ↔ Screw 6-32 x 0.500''-Silver:7
- [Mate]: 5 x 24:2 ↔ Screw 6-32 x 0.500''-Silver:8
- Mate:249: 2-Wire Motor 393-Without Wire:3 ↔ Screw 6-32 x 0.500''-Silver:8
- [Tangent] (0.4572 mm): 5 x 24:2 ↔ Screw 6-32 x 0.500''-Silver:6
- [Tangent] (0.4572 mm): 5 x 24:2 ↔ Screw 6-32 x 0.500''-Silver:6
- Mate:250: 5 x 24:2 ↔ Flat Bearing Block:11
- [Tangent] (0.4572 mm): 5 x 24:2 ↔ Screw 6-32 x 0.500''-Silver:5
- [Mate]: Screw 6-32 x 0.500''-Silver:6 ↔ 2-Wire Motor 393-Without Wire:4
- [Mate]: Screw 6-32 x 0.500''-Silver:5 ↔ 2-Wire Motor 393-Without Wire:4
- [Tangent] (0.4572 mm): 5 x 24:1 ↔ Screw 6-32 x 0.500''-Silver:3
- [Tangent] (0.4572 mm): 5 x 24:1 ↔ Screw 6-32 x 0.500''-Silver:3
- [Tangent] (0.4572 mm): 5 x 24:1 ↔ Screw 6-32 x 0.500''-Silver:4
- Mate:253: 5 x 24:1 ↔ 1103 Custom Chassis:1
- Mate:254: 5 x 24:1 ↔ 2 x 6:2
- Flush:18: 5 x 25:2 ↔ 2 x 6:2
- Flush:19: 5 x 25:2 ↔ 2 x 6:2
- Mate:255: 5 x 25:2 ↔ 2 x 6:1
- Flush:20: 5 x 25:2 ↔ 2 x 6:1
- Flush:21: 5 x 25:2 ↔ 2 x 6:1
- Flush:22: 5 x 25:2 ↔ 1103 Custom Chassis:1
- Flush:23: 5 x 25:2 ↔ 1103 Custom Chassis:1
- Flush:34: 5 x 24:2 ↔ 2 x 25:1
- [Mate]: 5 x 24:1 ↔ Standoff 0.50'':9
- [Mate]: 5 x 24:1 ↔ Standoff 0.50'':10
- [Tangent] (0.2286 mm): 5 x 24:1 ↔ Standoff 0.50'':9
- [Tangent] (0.2286 mm): 5 x 24:1 ↔ Standoff 0.50'':9
- [Tangent] (0.2286 mm): 5 x 24:1 ↔ Standoff 0.50'':10
- [Tangent] (0.2286 mm): 5 x 24:1 ↔ Standoff 0.50'':10
- [Mate]: Standoff 0.50'':9 ↔ 4 Slotted Angle:1
- [Tangent] (0.2286 mm): Standoff 0.50'':10 ↔ 4 Slotted Angle:1
- [Tangent] (0.2286 mm): Standoff 0.50'':9 ↔ 4 Slotted Angle:1
- [Tangent] (0.2286 mm): Standoff 0.50'':10 ↔ 4 Slotted Angle:1
- [Mate]: 4 Slotted Angle:1 ↔ Spacer (Nylon), 0.375'':1
- [Tangent]: 4 Slotted Angle:1 ↔ Spacer (Nylon), 0.375'':1
- [Tangent]: 4 Slotted Angle:1 ↔ Spacer (Nylon), 0.375'':1
- [Mate]: 4 Slotted Angle:1 ↔ Spacer (Nylon), 0.375'':2
- [Tangent]: 4 Slotted Angle:1 ↔ Spacer (Nylon), 0.375'':2
- [Tangent]: 4 Slotted Angle:1 ↔ Spacer (Nylon), 0.375'':2
- [Tangent] (0.2286 mm): Standoff 0.50'':2 ↔ 2 x 6:4
- [Tangent] (0.2286 mm): Standoff 0.50'':2 ↔ 2 x 6:4
- [Mate]: Standoff 0.50'':2 ↔ 2 x 6:4
- [Tangent] (0.2286 mm): 5 x 25:4 ↔ Standoff 0.50'':1
- [Tangent] (0.2286 mm): 5 x 25:4 ↔ Standoff 0.50'':1
- [Mate]: Standoff 0.50'':4 ↔ 2 x 6:4
- [Tangent] (0.2286 mm): Standoff 0.50'':4 ↔ 2 x 6:4
- [Tangent] (0.2286 mm): Standoff 0.50'':4 ↔ 2 x 6:4
- [Tangent] (0.2286 mm): 5 x 25:4 ↔ Standoff 0.50'':4
- [Tangent] (0.2286 mm): 5 x 25:4 ↔ Standoff 0.50'':4
- [Tangent] (0.2286 mm): 5 x 24:2 ↔ Standoff 0.50'':2
- [Tangent] (0.2286 mm): 5 x 24:2 ↔ Standoff 0.50'':3
- [Tangent] (0.2286 mm): 5 x 24:2 ↔ Standoff 0.50'':3
- [Mate]: Standoff 0.50'':1 ↔ 2 x 6:3
- [Tangent] (0.2286 mm): Standoff 0.50'':1 ↔ 2 x 6:3
- [Tangent] (0.2286 mm): Standoff 0.50'':1 ↔ 2 x 6:3
- [Tangent] (0.2286 mm): Standoff 0.50'':3 ↔ 2 x 6:3
- [Tangent] (0.2286 mm): Standoff 0.50'':6 ↔ 2 x 6:2
- [Tangent] (0.2286 mm): Standoff 0.50'':6 ↔ 2 x 6:2
- [Tangent] (0.2286 mm): Standoff 0.50'':7 ↔ 2 x 6:2
- [Tangent] (0.2286 mm): Standoff 0.50'':7 ↔ 2 x 6:2
- [Tangent] (0.2286 mm): Standoff 0.50'':5 ↔ 2 x 6:1
- [Tangent] (0.2286 mm): Standoff 0.50'':5 ↔ 2 x 6:1
- [Tangent] (0.2286 mm): Standoff 0.50'':8 ↔ 2 x 6:1
- [Tangent] (0.2286 mm): Standoff 0.50'':8 ↔ 2 x 6:1
- [Mate]: Spacer (Nylon), 0.375'':1 ↔ 4 x 6 cut:1
- [Tangent]: Spacer (Nylon), 0.375'':2 ↔ 4 x 6 cut:1
- [Tangent]: Spacer (Nylon), 0.375'':2 ↔ 4 x 6 cut:1
- [Tangent]: Spacer (Nylon), 0.375'':1 ↔ 4 x 6 cut:1
- [Flush]: 4 x 6 cut:1 ↔ Ultrasonic Range Finder (Sensor):1
- [Tangent] (-3.556 mm): 4 x 6 cut:1 ↔ Ultrasonic Range Finder (Sensor):1
- [Mate]: 5 x 24:2 ↔ Standoff 0.50'':11
- [Mate]: 5 x 24:2 ↔ Standoff 0.50'':12
- [Tangent] (0.2286 mm): 5 x 24:2 ↔ Standoff 0.50'':11
- [Tangent] (0.2286 mm): 5 x 24:2 ↔ Standoff 0.50'':11
- [Tangent] (0.2286 mm): 5 x 24:2 ↔ Standoff 0.50'':12
- [Tangent] (0.2286 mm): 5 x 24:2 ↔ Standoff 0.50'':12
- [Mate]: Standoff 0.50'':11 ↔ 4 Slotted Angle:2
- [Tangent] (0.2286 mm): Standoff 0.50'':11 ↔ 4 Slotted Angle:2
- [Tangent] (0.2286 mm): Standoff 0.50'':11 ↔ 4 Slotted Angle:2
- [Tangent] (0.2286 mm): Standoff 0.50'':12 ↔ 4 Slotted Angle:2
- [Mate]: 4 Slotted Angle:2 ↔ Spacer (Nylon), 0.375'':3
- [Mate]: 4 Slotted Angle:2 ↔ Spacer (Nylon), 0.375'':4
- [Tangent]: 4 Slotted Angle:2 ↔ Spacer (Nylon), 0.375'':4
- [Tangent]: 4 Slotted Angle:2 ↔ Spacer (Nylon), 0.375'':4
- [Tangent]: 4 Slotted Angle:2 ↔ Spacer (Nylon), 0.375'':3
- [Tangent]: 4 Slotted Angle:2 ↔ Spacer (Nylon), 0.375'':3
- [Mate]: Spacer (Nylon), 0.375'':3 ↔ 4 x 6 cut:2
- [Tangent]: Spacer (Nylon), 0.375'':3 ↔ 4 x 6 cut:2
- [Tangent]: Spacer (Nylon), 0.375'':3 ↔ 4 x 6 cut:2
- [Tangent]: Spacer (Nylon), 0.375'':4 ↔ 4 x 6 cut:2
- [Flush]: 4 x 6 cut:2 ↔ Ultrasonic Range Finder (Sensor):2
- [Tangent]: 4 x 6 cut:2 ↔ Ultrasonic Range Finder (Sensor):2
- [Mate]: 5 x 24:2 ↔ Screw 8-32 x 0.500''-Silver:8
- Rotation:2 [RelateRotation] (1 ul): 5 x 25:4 ↔ Flat Bearing Block:15
- Flush:56: 5 x 25:4 ↔ 1103 Custom Chassis:1
- Flush:57: 5 x 24:2 ↔ 2 x 6:3
- Mate:318: 5 x 24:1 ↔ Bearing Block:4
- Flush:58: 5 x 25:2 ↔ 5 x 24:1
- Flush:59: 5 x 25:2 ↔ 5 x 24:1
- Mate:319: Flat Bearing Block:7 ↔ .5'' Screw & Nylock Nut:1
- Mate:320: Flat Bearing Block:7 ↔ .5'' Screw & Nylock Nut:1
- Mate:322: 5 x 24:1 ↔ .5'' Screw & Nylock Nut:2
- Mate:323: Flat Bearing Block:7 ↔ .5'' Screw & Nylock Nut:2
- Mate:324: Flat Bearing Block:1 ↔ 2x .5'' Screw & Nylock Nut:1
- Mate:325: Flat Bearing Block:1 ↔ 2x .5'' Screw & Nylock Nut:1
- Mate:326: 5 x 25:2 ↔ 2x .5'' Screw & Nylock Nut:1
- Mate:327: 5 x 25:2 ↔ .5'' Screw & Nylock Nut:3
- Mate:328: .5'' Screw & Nylock Nut:3 ↔ Flat Bearing Block:2
- Mate:329: Flat Bearing Block:2 ↔ .5'' Screw & Nylock Nut:4
- Mate:330: 5 x 25:2 ↔ .5'' Screw & Nylock Nut:4
- Tangent:152 (0.2311 mm): 5 x 24:1 ↔ Bearing Block:1
- Tangent:153 (0.2311 mm): 5 x 24:1 ↔ Bearing Block:1
- Tangent:154 (0.2311 mm): 5 x 24:1 ↔ Bearing Block:1
- Tangent:155 (0.2311 mm): 5 x 24:1 ↔ Bearing Block:4
- Tangent:156 (0.2311 mm): 5 x 24:1 ↔ Bearing Block:4
- Tangent:157 (0.2311 mm): 5 x 24:2 ↔ Bearing Block:2
- Tangent:158 (0.2311 mm): 5 x 24:2 ↔ Bearing Block:2
- Tangent:159 (0.2311 mm): 5 x 24:2 ↔ Bearing Block:2
- Tangent:160 (0.2311 mm): 5 x 24:2 ↔ Bearing Block:3
- Tangent:161 (0.2311 mm): 5 x 24:2 ↔ Bearing Block:3
- Tangent:162 (0.2311 mm): 5 x 24:2 ↔ Bearing Block:3
- Mate:332: .5'' Screw & Nylock Nut:5 ↔ Flat Bearing Block:10
- Mate:333: 5 x 24:2 ↔ .5'' Screw & Nylock Nut:5
- Mate:334: Flat Bearing Block:10 ↔ Nut 8-32 Nylock:1
- Mate:335: Screw 8-32 x 0.500''-Silver:8 ↔ Nut 8-32 Nylock:1
- Mate:336: Screw 8-32 x 0.500''-Silver:17 ↔ Nut 8-32 Nylock:2
- Mate:337: Screw 8-32 x 0.500''-Silver:18 ↔ Nut 8-32 Nylock:3
- Mate:338: Flat Bearing Block:17 ↔ Nut 8-32 Nylock:2
- Mate:339: Flat Bearing Block:17 ↔ Nut 8-32 Nylock:3
- Mate:340: Flat Bearing Block:16 ↔ Nut 8-32 Nylock:4
- Mate:341: Flat Bearing Block:16 ↔ Nut 8-32 Nylock:5
- Mate:342: Screw 8-32 x 0.500''-Silver:15 ↔ Nut 8-32 Nylock:4
- Mate:343: Screw 8-32 x 0.500''-Silver:16 ↔ Nut 8-32 Nylock:5
- Mate:344: Flat Bearing Block:14 ↔ Nut 8-32 Nylock:7
- Mate:345: Flat Bearing Block:14 ↔ Nut 8-32 Nylock:6
- Mate:346: Screw 8-32 x 0.500''-Silver:11 ↔ Nut 8-32 Nylock:7
- Mate:347: Screw 8-32 x 0.500''-Silver:12 ↔ Nut 8-32 Nylock:6
- Mate:348: Flat Bearing Block:15 ↔ Nut 8-32 Nylock:8